# Autodesk Inventor assembly: 6409
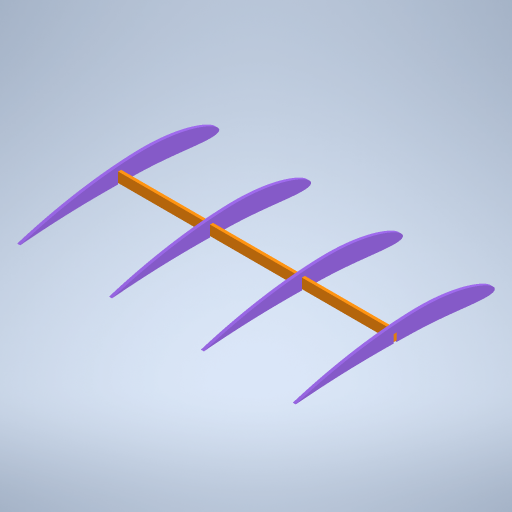
[picture p0: Inventor's stored thumbnail of the model, 512x512]
Saved by Autodesk Inventor 2023 (Build 270158000, 158)
## iProperties
Created: 2023-03-24
Part Number: 6409
Document SubType Name: Assembly
Designer: USER
Author: USER
## Documents named in this file (3)
- D:\Github Download\ME_project\Areo_Rider_Cabin\Airfoil & Nuzzle\airfoil_v2\6409.iam
- D:\Github Download\ME_project\Areo_Rider_Cabin\Airfoil & Nuzzle\airfoil_v2\支撐架.ipt
- D:\Github Download\ME_project\Areo_Rider_Cabin\Airfoil & Nuzzle\airfoil_v2\6409_v1.ipt
## Components (5 placed, 2 different names)
1. 支撐架:1 — 貼合:1, 貼合:2, 貼合:3, 貼合:4, 貼合:5, 貼合:6, 貼合:7, 貼合:8, 貼合:9, 貼合:10, 貼合:11, 貼合:12
2. 6409_v1:1 — 貼合:1, 貼合:5, 貼合:9
3. 6409_v1:2 — 貼合:2, 貼合:6, 貼合:10
4. 6409_v1:3 — 貼合:3, 貼合:7, 貼合:11
5. 6409_v1:4 — 貼合:4, 貼合:8, 貼合:12
## Relationships (12: Mate 12)
- 貼合:1 [Mate]: 支撐架:1 ↔ 6409_v1:1
- 貼合:2 [Mate]: 支撐架:1 ↔ 6409_v1:2
- 貼合:3 [Mate]: 支撐架:1 ↔ 6409_v1:3
- 貼合:4 [Mate]: 支撐架:1 ↔ 6409_v1:4
- 貼合:5 [Mate]: 支撐架:1 ↔ 6409_v1:1
- 貼合:6 [Mate]: 支撐架:1 ↔ 6409_v1:2
- 貼合:7 [Mate]: 支撐架:1 ↔ 6409_v1:3
- 貼合:8 [Mate]: 支撐架:1 ↔ 6409_v1:4
- 貼合:9 [Mate]: 支撐架:1 ↔ 6409_v1:1
- 貼合:10 [Mate]: 支撐架:1 ↔ 6409_v1:2
- 貼合:11 [Mate]: 支撐架:1 ↔ 6409_v1:3
- 貼合:12 [Mate]: 支撐架:1 ↔ 6409_v1:4
